# Autodesk Inventor assembly: Base
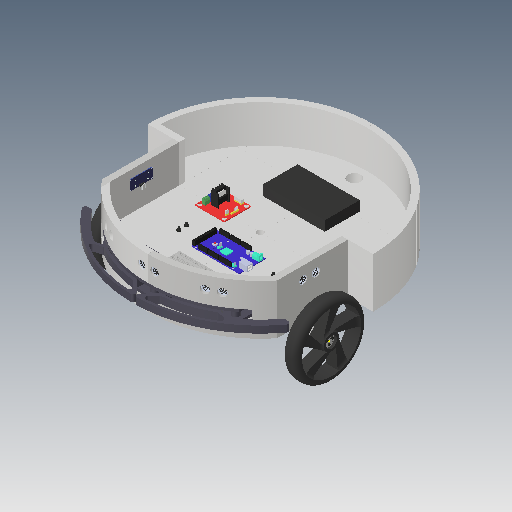
[picture p0: Inventor's stored thumbnail of the model, 512x512]
Saved by Autodesk Inventor 2017 (Build 210142000, 142)
## iProperties
Created: 2017-03-11
Part Number: Base
Document SubType Name: Assembly
Designer: zallen
Author: zallen
## Documents named in this file (18)
- C:\Users\zallen\Documents\GitHub\cr-laundry-robot\src\Base\Base.iam
- C:\Users\zallen\Documents\GitHub\cr-laundry-robot\src\Base\Chassis.ipt
- C:\Users\zallen\Documents\GitHub\cr-laundry-robot\src\Base\Swivel Wheel.ipt
- C:\Users\zallen\Documents\Autodesk Inventor Projects\HC-SR04 Ultasonic Sensor\Sensor Ultrasónico.ipt
- C:\Users\zallen\Documents\Autodesk Inventor Projects\Breadboard\breadboard_350_pos_asm.iam
- C:\Users\zallen\Documents\Autodesk Inventor Projects\Arduino Mega 2560\Arduino Mega 2560.ipt
- C:\Users\zallen\Documents\Autodesk Inventor Projects\L298n\Драйвер двигателей L298N.ipt
- C:\Users\zallen\Documents\GitHub\cr-laundry-robot\src\Base\Drive Wheel Assembly\DriveAssembly.iam
- C:\Users\zallen\Documents\GitHub\cr-laundry-robot\src\Base\Design Accelerator\Bolted Connection2.iam
- C:\Users\zallen\Documents\GitHub\cr-laundry-robot\src\Base\Design Accelerator\Bolted Connection3.iam
- C:\Users\zallen\Documents\GitHub\cr-laundry-robot\src\Base\Design Accelerator\Bolted Connection4.iam
- C:\Users\zallen\Documents\GitHub\cr-laundry-robot\src\Base\Design Accelerator\Bolted Connection5.iam
- C:\Users\zallen\Documents\GitHub\cr-laundry-robot\src\Base\Battery Pack Assembly\BatteryPackAssembly.iam
- C:\Users\zallen\Documents\GitHub\cr-laundry-robot\src\Base\Bumper Assembly\Bumper Assembly.iam
- C:\Users\zallen\Documents\GitHub\cr-laundry-robot\src\Base\Base\Design Accelerator\Bolted Connection1.iam
- C:\Users\zallen\Documents\GitHub\cr-laundry-robot\src\Base\Base\Design Accelerator\Bolted Connection2.iam
- C:\Users\zallen\Documents\GitHub\cr-laundry-robot\src\Base\Base\Design Accelerator\Bolted Connection3.iam
- C:\Users\zallen\Documents\GitHub\cr-laundry-robot\src\Base\Base\Design Accelerator\Bolted Connection4.iam
## Components (21 placed, 10 different names)
1. Chassis:1 — Mate:22, Mate:23, Mate:24, Mate:25, Mate:26, Mate:27, Mate:28, Mate:29, Mate:31, Mate:32, Mate:33, Mate:36, Mate:37, Mate:38, Mate:39, Mate:40, Mate:41, Mate:42, Mate:43, Mate:44, Mate:45, Mate:46, Mate:55, Mate:56, Mate:57
2. Swivel Wheel:1 — Mate:22, Mate:23
3. Sensor Ultrasónico:1 — Mate:24, Mate:29
4. Sensor Ultrasónico:2 — Mate:25, Mate:27
5. Sensor Ultrasónico:3 — Mate:26, Mate:28
6. breadboard_350_pos_asm:1 [sub-assembly] — Mate:31
7. Arduino Mega 2560:1 — Mate:32
8. L298N:1 — Mate:33
9. Sensor Ultrasónico:4 — Mate:36, Mate:37, Mate:38
10. Sensor Ultrasónico:5 — Mate:39, Mate:40, Mate:41
11. DriveAssembly:1 [sub-assembly] — Mate:42, Mate:43, Mate:44, Mate:45, Mate:46, Mate:47, Mate:48, Mate:49, Mate:50, Mate:51, Mate:52, Mate:53, Mate:54
12. Bolted Connection:1 [sub-assembly] — Mate:47, Mate:48
13. Bolted Connection:2 [sub-assembly] — Mate:49, Mate:50
14. Bolted Connection:3 [sub-assembly] — Mate:51, Mate:52
15. Bolted Connection:4 [sub-assembly] — Mate:53, Mate:54
16. BatteryPackAssembly:1 [sub-assembly] — Mate:55
17. Bumper Assembly:1 [sub-assembly] — Mate:56, Mate:57, Mate:58, Mate:59, Mate:60, Mate:61, Mate:62, Mate:63, Mate:64, Mate:65
18. Bolted Connection:5 [sub-assembly] — Mate:58, Mate:59
19. Bolted Connection:6 [sub-assembly] — Mate:60, Mate:61
20. Bolted Connection:7 [sub-assembly] — Mate:62, Mate:63
21. Bolted Connection:8 [sub-assembly] — Mate:64, Mate:65
## Relationships (41: Mate 41)
- Mate:22: Chassis:1 ↔ Swivel Wheel:1
- Mate:23: Chassis:1 ↔ Swivel Wheel:1
- Mate:24: Chassis:1 ↔ Sensor Ultrasónico:1
- Mate:25: Chassis:1 ↔ Sensor Ultrasónico:2
- Mate:26: Chassis:1 ↔ Sensor Ultrasónico:3
- Mate:27: Chassis:1 ↔ Sensor Ultrasónico:2
- Mate:28: Chassis:1 ↔ Sensor Ultrasónico:3
- Mate:29: Chassis:1 ↔ Sensor Ultrasónico:1
- Mate:31: Chassis:1 ↔ breadboard_350_pos_asm:1
- Mate:32: Chassis:1 ↔ Arduino Mega 2560:1
- Mate:33: Chassis:1 ↔ L298N:1
- Mate:36: Chassis:1 ↔ Sensor Ultrasónico:4
- Mate:37: Chassis:1 ↔ Sensor Ultrasónico:4
- Mate:38: Chassis:1 ↔ Sensor Ultrasónico:4
- Mate:39: Chassis:1 ↔ Sensor Ultrasónico:5
- Mate:40: Chassis:1 ↔ Sensor Ultrasónico:5
- Mate:41: Chassis:1 ↔ Sensor Ultrasónico:5
- Mate:42: Chassis:1 ↔ DriveAssembly:1
- Mate:43: Chassis:1 ↔ DriveAssembly:1
- Mate:44: Chassis:1 ↔ DriveAssembly:1
- Mate:45: Chassis:1 ↔ DriveAssembly:1
- Mate:46: Chassis:1 ↔ DriveAssembly:1
- Mate:47: DriveAssembly:1 ↔ Bolted Connection:1
- Mate:48: DriveAssembly:1 ↔ Bolted Connection:1
- Mate:49: DriveAssembly:1 ↔ Bolted Connection:2
- Mate:50: DriveAssembly:1 ↔ Bolted Connection:2
- Mate:51: DriveAssembly:1 ↔ Bolted Connection:3
- Mate:52: DriveAssembly:1 ↔ Bolted Connection:3
- Mate:53: DriveAssembly:1 ↔ Bolted Connection:4
- Mate:54: DriveAssembly:1 ↔ Bolted Connection:4
- Mate:55: Chassis:1 ↔ BatteryPackAssembly:1
- Mate:56: Chassis:1 ↔ Bumper Assembly:1
- Mate:57: Chassis:1 ↔ Bumper Assembly:1
- Mate:58: Bumper Assembly:1 ↔ Bolted Connection:5
- Mate:59: Bumper Assembly:1 ↔ Bolted Connection:5
- Mate:60: Bumper Assembly:1 ↔ Bolted Connection:6
- Mate:61: Bumper Assembly:1 ↔ Bolted Connection:6
- Mate:62: Bumper Assembly:1 ↔ Bolted Connection:7
- Mate:63: Bumper Assembly:1 ↔ Bolted Connection:7
- Mate:64: Bumper Assembly:1 ↔ Bolted Connection:8
- Mate:65: Bumper Assembly:1 ↔ Bolted Connection:8
